# Autodesk Inventor assembly: SSEBZ-MX10-55
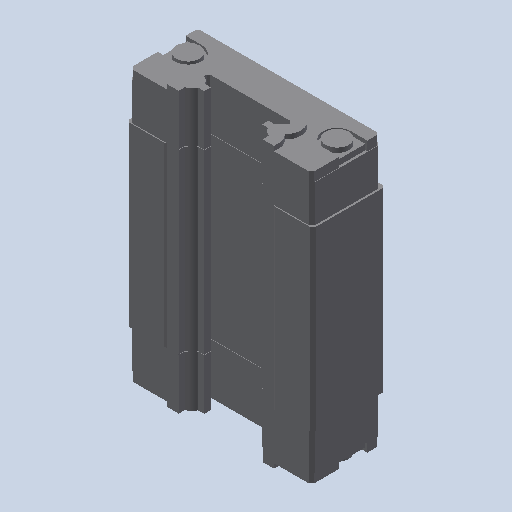
[picture p0: Inventor's stored thumbnail of the model, 512x512]
Saved by Autodesk Inventor 2025.1 (Build 291241000, 241)
## iProperties
Category: PARTsolutions
Company: MISUMI
Created: 2022-11-22
Part Number: SSEBZ-MX10-55
Catalog Web Link: www.cadenas.de
Description: SSEBZ, SSEBZ-MX, SSE2BZ, SSE2BZ-MX-Miniature Slide Guides Standard/Interchangeable, Small Clearance Standard Selectable Type
Vendor: MISUMI
Document SubType Name: Assembly
Designer: psAdmin
Manufacturer: MISUMI
Mass: 5.67333 g
Surface Area: 44.6338 cm^2
Volume: 5.67333 cm^3
PSOL_IDENT_0: {$CADENAS_DATA/23d-libs/misumi/metric/06_linear_guides/sebz_asmtab.prj},246 {VTYP=3D},{STYP=ASSTAB},
PSOL_IDENT_1: {NB=SSEBZ-MX10-55},{LINA=SSEBZ-MX10-55},{NN=SSEBZ, SSEBZ-MX, SSE2BZ, SSE2BZ-MX},{DATE=17.06.2022 02:
PSOL_IDENT_2: 33:09},{GEOMDATE=16.06.2022 00:46:50},{VERSION=},{LINEID=160},{WBVAR=MAT,MX,NOB,GREASE,LS,ALT1,ALT2,
PSOL_IDENT_3: ALT4},{WBNUMERIC=LS}  {NB=SSEBZ-MX10-55},{LINA=SSEBZ-MX10-55},{KT=DUMMY},{PN=SSEBZ-MX10-55},{RT=B},{
PSOL_IDENT_4: TYPE=SSEBZ},{MAT=S},{MX=-MX},{MXALG='', 'w/o MX(Lubrication unit)', '-MX', 'with MX(Lubrication unit
PSOL_IDENT_5: )'},{NOB=},{H=10},{GREASE=},{GREASEALG='','Normal'},{LT=Selectable},{LS=55},{W=20},{L1=30.0},{B=15},
PSOL_IDENT_6: {C=10},{SLL=M3x3},{L2=19.0},{K=7.8},{CBB=0.3},{W1=9},{W2=5.5},{H1=5.5},{CAA=0.3},{DD1DD2HH=3.5x6x3.5
PSOL_IDENT_7: },{F=20},{G=7.5},{ALT1=},{ALT1ALG= '', 'w/o MC (Tapped Holes)', '-MC', 'with MC (Tapped Holes)' },{M
PSOL_IDENT_8: C=M4},{ALT2=},{ALT2L=2.5},{ALT2N=5},{M=3},{LL=},{L0=35,55,75,95,115,135,155,175,195,215,235,255,275,
PSOL_IDENT_9: 295,315,335,355,355,375,395,415,435,455,475,495,515,535,555,575,595,615,635},{REC1=   '','w/o Rail E
PSOL_IDENT_10: nds Cut alteration','-LLC','with LLC (Left End Cut)','-RLC','with RLC (Right End Cut)','-LLC-RLC','w
PSOL_IDENT_11: ith Both End Cut'   },{MAT2='S','Stainless Steel'},{ALT4=},{ALT4ALG= '','Not applicable' },{PPATH=ss
PSOL_IDENT_12: ebz_series/sebz_asmtpl.prj}
NB: SSEBZ-MX10-55
NN: SSEBZ, SSEBZ-MX, SSE2BZ, SSE2BZ-MX
NT: Miniature Slide Guides Standard/Interchangeable, Small Clearance Standard Selectable Type
NBSYN: $PN.
LINA: SSEBZ-MX10-55
CATALOG: Misumi
PN: SSEBZ-MX10-55
MAT: Stainless Steel
MX: with MX(Lubrication unit)
NOB: 1
H: 10
GREASE: Normal
LS: 55
W: 20
L1: 30
B: 15
C: 10
SLL: M3x3
L2: 19
K: 7.8
CBB: 0.3
W1: 9
W2: 5.5
H1: 5.5
CAA: 0.3
DD1DD2HH: 3.5x6x3.5
F: 20
G: 7.5
ALT1: w/o MC (Tapped Holes)
ALT2: w/o Rail Ends Cut alteration
ALT4: Not applicable
SUPPLIER: MISUMI
ARTICLENO: SSEBZ-MX10-55
BOMINFO: SSEBZ-MX10-55
CREATOR: CADENAS GmbH
Title: SSEBZ-MX10-55
Author: Cadenas PARTsolutions
Comments: Miniature Slide Guides Standard/Interchangeable, Small Clearance Standard Selectable Type
## Documents named in this file (3)
- C:\Users\haruy\Documents\ロボコン\NHK2025\cad\000_parts\スライダー\SSEBZ-MX10-55.iam
- C:\Users\haruy\OneDrive - Kyushu University\KURT_工房共有\2023~2024\ハード\CAD\2024NHK\nagahisa\R1\touteki\SSEBZ-MX10-55_r.ipt
- C:\Users\haruy\Documents\ロボコン\NHK2025\cad\nagahisa\hand\grab\SSEBZ-MX10_b.ipt
## Components (2 placed, 2 different names)
1. SSEBZ-MX10-55_r:1 — to_block_Z@1 <-> to_rail_Z@2, to_block_YZ@1 <-> to_rail_YZ@2
2. SSEBZ-MX10_b:1 — to_block_Z@1 <-> to_rail_Z@2, to_block_YZ@1 <-> to_rail_YZ@2
## Relationships (2: Mate 1, Angle 1)
- to_block_Z@1 <-> to_rail_Z@2 [Mate]: SSEBZ-MX10-55_r:1 ↔ SSEBZ-MX10_b:1
- to_block_YZ@1 <-> to_rail_YZ@2 [Angle] (0 deg): SSEBZ-MX10-55_r:1 ↔ SSEBZ-MX10_b:1
